# Autodesk Inventor assembly: Schalter_0-100
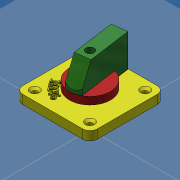
[picture p0: Inventor's stored thumbnail of the model, 180x180]
Saved by Autodesk Inventor 2019 (Build 230136000, 136)
## iProperties
Created: 2020-08-07
Part Number: Schalter_0-100
Material: Generisch
Document SubType Name: Assembly
Designer: Stefan
Mass: 23.836 g
Surface Area: 121.346 cm^2
Volume: 23.836 cm^3
Density: 1 g/cm^3
Author: Stefan
## Documents named in this file (4)
- C:\Users\User\OneDrive\Dokumente\Inventor\Absauganlage\Schalter_0-100.iam
- C:\Users\User\OneDrive\Dokumente\Inventor\Absauganlage\Schalter_Platte_0-100.ipt
- C:\Users\User\OneDrive\Dokumente\Inventor\Absauganlage\Schalter_Knauf.ipt
- C:\Users\User\OneDrive\Dokumente\Inventor\Absauganlage\Schalter_Basis_rund.ipt
## Components (3 placed, 3 different names)
1. Schalter_Platte_0-100:1 — Passend:4, Passend:5
2. Schalter_Knauf:1 — Passend:1, Passend:2, Passend:3
3. Schalter_Basis_rund:1 — Passend:1, Passend:2, Passend:3, Passend:4, Passend:5
## Relationships (5: Mate 5)
- Passend:1 [Mate]: Schalter_Knauf:1 ↔ Schalter_Basis_rund:1
- Passend:2 [Mate]: Schalter_Knauf:1 ↔ Schalter_Basis_rund:1
- Passend:3 [Mate]: Schalter_Knauf:1 ↔ Schalter_Basis_rund:1
- Passend:4 [Mate]: Schalter_Platte_0-100:1 ↔ Schalter_Basis_rund:1
- Passend:5 [Mate]: Schalter_Platte_0-100:1 ↔ Schalter_Basis_rund:1
